# Autodesk Inventor assembly: mainASM
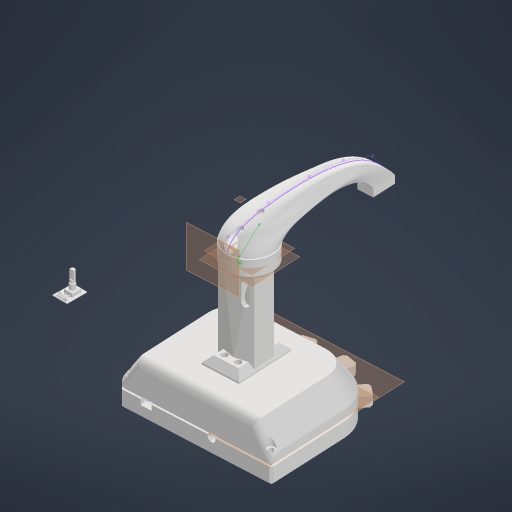
[picture p0: Inventor's stored thumbnail of the model, 512x512]
Saved by Autodesk Inventor 2024 (Build 280153000, 153)
## iProperties
Created: 2024-03-11
Part Number: mainASM
Document SubType Name: Assembly
Designer: Daniel
Author: Daniel
## Documents named in this file (12)
- C:\Users\Daniel\Desktop\pmik_2024l_jd\mechanical\mainASM.iam
- C:\Users\Daniel\Desktop\pmik_2024l_jd\mechanical\STEPS\NUCLEO-F091RC.iam
- C:\Users\Daniel\Desktop\pmik_2024l_jd\mechanical\STEPS\SG90 - Micro Servo 9g - Tower Pro.iam
- C:\Users\Daniel\Desktop\pmik_2024l_jd\mechanical\STEPS\KY-040 Rotary Encoder.iam
- C:\Users\Daniel\Desktop\pmik_2024l_jd\mechanical\bottom.ipt
- C:\Users\Daniel\Desktop\pmik_2024l_jd\mechanical\Pump.ipt
- C:\Users\Daniel\Desktop\pmik_2024l_jd\mechanical\STEPS\LM2596 DC to DC Buck Converter 3 A.iam
- C:\Users\Daniel\Desktop\pmik_2024l_jd\mechanical\Top.ipt
- C:\Users\Daniel\Desktop\pmik_2024l_jd\mechanical\Tower.ipt
- C:\Users\Daniel\Documents\Inventor\Content Center Files\R2024\pl-PL\M\M 4x30.ipt
- C:\Users\Daniel\Documents\Inventor\Content Center Files\R2024\pl-PL\M\M 3x10.ipt
- C:\Users\Daniel\Desktop\pmik_2024l_jd\mechanical\Head.ipt
## Components (20 placed, 11 different names)
1. NUCLEO-F091RC:1 [sub-assembly] — Mate:3, Mate:4, Mate:5, Rotational:5, Rotational:6
2. SG90 - Micro Servo 9g - Tower Pro:1 [sub-assembly] — Mate:10, Flush:11, Flush:12
3. KY-040 Rotary Encoder:1 [sub-assembly]
4. bottom:1 — Flush:1, Angle:1, Mate:3, Mate:4, Mate:5, Mate:6, Mate:7, Mate:8, Mate:9, Flush:2, Flush:3, Flush:4, Flush:5, Flush:8
5. Pump:1 — Angle:1, Mate:6, Mate:7, Mate:8
6. LM2596 DC to DC Buck Converter 3 A:1 [sub-assembly] — Mate:9, Flush:2, Flush:3, Rotational:3, Rotational:4
7. Top:1 — Flush:4, Flush:5, Rotational:1, Rotational:2, Rigid:1, Flush:6, Flush:7, Flush:8
8. M 4x30:12 — Rotational:2
9. M 4x30:13 — Rigid:1
10. M 4x30:14 — Rotational:1
11. M 3x10:5 — Rotational:4
12. M 3x10:6 — Rotational:3
13. M 3x10:7 — Rotational:5
14. M 3x10:8 — Rotational:6
15. Tower:1 — Flush:6, Flush:7, Rotational:7, Rotational:8, Rotational:9, Rotational:10, Mate:10, Flush:9, Flush:10
16. M 4x30:8 — Rotational:7
17. M 4x30:9 — Rotational:8
18. M 4x30:10 — Rotational:9
19. M 4x30:11 — Rotational:10
20. Head:1 — Flush:9, Flush:10, Flush:11, Flush:12
## Relationships (32: Flush 12, RevoluteJoint 10, Mate 8, Angle 1, WeldJoint 1)
- Flush:1: bottom:1
- Angle:1 (180 deg): bottom:1 ↔ Pump:1
- Mate:3 (3 mm): NUCLEO-F091RC:1 ↔ bottom:1
- Mate:4 (2 mm): NUCLEO-F091RC:1 ↔ bottom:1
- Mate:5 (5 mm): NUCLEO-F091RC:1 ↔ bottom:1
- Mate:6 (25 mm): bottom:1 ↔ Pump:1
- Mate:7 (5 mm): bottom:1 ↔ Pump:1
- Mate:8 (3 mm): bottom:1 ↔ Pump:1
- Mate:9 (5 mm): bottom:1 ↔ LM2596 DC to DC Buck Converter 3 A:1
- Flush:2 (5 mm): bottom:1 ↔ LM2596 DC to DC Buck Converter 3 A:1
- Flush:3 (4 mm): bottom:1 ↔ LM2596 DC to DC Buck Converter 3 A:1
- Flush:4: bottom:1 ↔ Top:1
- Flush:5: bottom:1 ↔ Top:1
- Rotational:1 [RevoluteJoint]: Top:1 ↔ M 4x30:14
- Rotational:2 [RevoluteJoint]: Top:1 ↔ M 4x30:12
- Rigid:1 [WeldJoint]: Top:1 ↔ M 4x30:13
- Rotational:3 [RevoluteJoint]: LM2596 DC to DC Buck Converter 3 A:1 ↔ M 3x10:6
- Rotational:4 [RevoluteJoint]: LM2596 DC to DC Buck Converter 3 A:1 ↔ M 3x10:5
- Rotational:5 [RevoluteJoint]: NUCLEO-F091RC:1 ↔ M 3x10:7
- Rotational:6 [RevoluteJoint]: NUCLEO-F091RC:1 ↔ M 3x10:8
- Flush:6: Top:1 ↔ Tower:1
- Flush:7: Top:1 ↔ Tower:1
- Rotational:7 [RevoluteJoint]: Tower:1 ↔ M 4x30:8
- Rotational:8 [RevoluteJoint]: Tower:1 ↔ M 4x30:9
- Rotational:9 [RevoluteJoint]: Tower:1 ↔ M 4x30:10
- Rotational:10 [RevoluteJoint]: Tower:1 ↔ M 4x30:11
- Mate:10: SG90 - Micro Servo 9g - Tower Pro:1 ↔ Tower:1
- Flush:8: bottom:1 ↔ Top:1
- Flush:9: Tower:1 ↔ Head:1
- Flush:10: Tower:1 ↔ Head:1
- Flush:11: SG90 - Micro Servo 9g - Tower Pro:1 ↔ Head:1
- Flush:12: SG90 - Micro Servo 9g - Tower Pro:1 ↔ Head:1
